# Autodesk Inventor assembly: Ensamblaje1
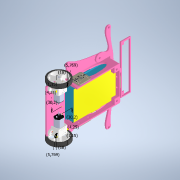
[picture p0: Inventor's stored thumbnail of the model, 180x180]
Saved by Autodesk Inventor 2021 (Build 250183000, 183)
## iProperties
Created: 2022-04-09
Part Number: Ensamblaje1
Document SubType Name: Assembly
Designer: skatl
Author: skatl
## Documents named in this file (8)
- C:\Users\skatl\Desktop\YO\CT2022\Cybertech2022\PRO_Loren\3D\Ensamblaje1.iam
- C:\Users\skatl\Desktop\YO\CT2022\Cybertech2022\PRO_Loren\3D\Body.ipt
- C:\Users\skatl\Desktop\YO\CT2022\Cybertech2022\PRO_Loren\3D\VL6180X - HiLetgo.ipt
- C:\Users\skatl\Desktop\YO\CT2022\Cybertech2022\PRO_Loren\3D\PCB_Tamaño.ipt
- C:\Users\skatl\Desktop\YO\CT2022\Cybertech2022\PRO_Loren\3D\VL6180X - HiLetgo.iam
- C:\Users\skatl\Desktop\YO\CT2022\Cybertech2022\PRO_Loren\3D\micro-metal-gearmotor-extended-with-1086-bracket.ipt
- C:\Users\skatl\Desktop\YO\CT2022\Cybertech2022\PRO_Loren\3D\pololu-wheel-32x7mm-white.ipt
- C:\Users\skatl\Desktop\YO\CT2022\Cybertech2022\PRO_Loren\3D\Siguelineas.ipt
## Components (11 placed, 6 different names)
1. Body:1 — Coincidencia:1, Coincidencia:2, Coincidencia:3, Insertar:3, Insertar:5, Insertar:8, Insertar:9, Insertar:11, Insertar:12
2. PCB_Tamaño:1 — Coincidencia:1, Coincidencia:2, Coincidencia:3
3. VL6180X - HiLetgo:3 [sub-assembly] — Insertar:3
4. micro-metal-gearmotor-extended-with-1086-bracket:1 — Insertar:5, Coincidencia:5, Insertar:7, Insertar:10
5. micro-metal-gearmotor-extended-with-1086-bracket:2 — Coincidencia:4, Insertar:6, Insertar:10
6. pololu-wheel-32x7mm-white:1 — Coincidencia:4, Insertar:6
7. pololu-wheel-32x7mm-white:2 — Coincidencia:5, Insertar:7
8. VL6180X - HiLetgo:5 — Insertar:9
9. VL6180X - HiLetgo:6 — Insertar:8
10. VL6180X - HiLetgo:7 — Insertar:11
11. Siguelineas:1 — Insertar:12
## Relationships (14: Insert 9, Mate 5)
- Coincidencia:1 [Mate]: Body:1 ↔ PCB_Tamaño:1
- Coincidencia:2 [Mate] (0.5 mm): Body:1 ↔ PCB_Tamaño:1
- Coincidencia:3 [Mate]: Body:1 ↔ PCB_Tamaño:1
- Insertar:3: Body:1 ↔ VL6180X - HiLetgo:3
- Insertar:5: Body:1 ↔ micro-metal-gearmotor-extended-with-1086-bracket:1
- Coincidencia:4 [Mate]: micro-metal-gearmotor-extended-with-1086-bracket:2 ↔ pololu-wheel-32x7mm-white:1
- Insertar:6: micro-metal-gearmotor-extended-with-1086-bracket:2 ↔ pololu-wheel-32x7mm-white:1
- Coincidencia:5 [Mate]: micro-metal-gearmotor-extended-with-1086-bracket:1 ↔ pololu-wheel-32x7mm-white:2
- Insertar:7: micro-metal-gearmotor-extended-with-1086-bracket:1 ↔ pololu-wheel-32x7mm-white:2
- Insertar:8: Body:1 ↔ VL6180X - HiLetgo:6
- Insertar:9: Body:1 ↔ VL6180X - HiLetgo:5
- Insertar:10 (10 mm): micro-metal-gearmotor-extended-with-1086-bracket:1 ↔ micro-metal-gearmotor-extended-with-1086-bracket:2
- Insertar:11: Body:1 ↔ VL6180X - HiLetgo:7
- Insertar:12: Body:1 ↔ Siguelineas:1
